# Autodesk Inventor assembly: お盆試作2
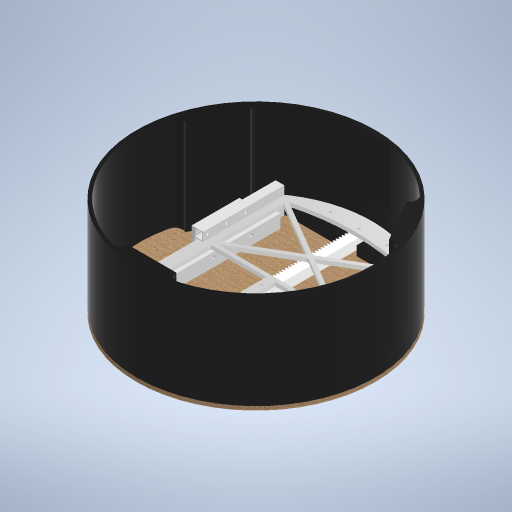
[picture p0: Inventor's stored thumbnail of the model, 512x512]
Saved by Autodesk Inventor 2023 (Build 270158000, 158)
## iProperties
Created: 2022-12-04
Part Number: お盆試作2
Document SubType Name: Assembly
Designer: RiSA
Author: RiSA
## Documents named in this file (9)
- E:\ロボ創\お盆試作2\お盆試作2.iam
- E:\ロボ創\お盆試作2\中間台1.ipt
- E:\ロボ創\お盆試作2\lock1.ipt
- E:\ロボ創\お盆試作2\lock2.ipt
- E:\ロボ創\お盆試作2\allwall.ipt
- E:\ロボ創\お盆試作2\slider.ipt
- E:\ロボ創\お盆試作2\お盆完成予定1.iam
- E:\ロボ創\お盆試作2\stopper.ipt
- E:\ロボ創\お盆試作2\squareEx1.ipt
## Components (11 placed, 8 different names)
1. 中間台1:1 — メイト:1, メイト:2, メイト:3, メイト:4, メイト:5, メイト:6, メイト:7, メイト:8
2. lock1:2 — メイト:1, メイト:2, メイト:3, メイト:9, メイト:10, メイト:11, フラッシュ:1, フラッシュ:2, メイト:19, メイト:20, メイト:21
3. lock2:1 — メイト:4, メイト:5, メイト:6, メイト:12, メイト:13, メイト:14, メイト:16, メイト:17, メイト:18
4. allwall:1 — メイト:7, メイト:8
5. slider:1 — メイト:9, メイト:10, メイト:11
6. slider:2 — メイト:12, メイト:13, メイト:14, メイト:15
7. お盆完成予定1:1 [sub-assembly] — メイト:15, フラッシュ:1, フラッシュ:2
8. stopper:1 — メイト:16, メイト:17, メイト:18, メイト:25, メイト:26
9. stopper:2 — メイト:19, メイト:20, メイト:21, メイト:22, メイト:23, メイト:24
10. squareEx1:1 — メイト:22, メイト:23, メイト:24
11. squareEx1:2 — メイト:25, メイト:26
## Relationships (28: Mate 26, Flush 2)
- メイト:1 [Mate]: 中間台1:1 ↔ lock1:2
- メイト:2 [Mate]: 中間台1:1 ↔ lock1:2
- メイト:3 [Mate]: 中間台1:1 ↔ lock1:2
- メイト:4 [Mate]: 中間台1:1 ↔ lock2:1
- メイト:5 [Mate]: 中間台1:1 ↔ lock2:1
- メイト:6 [Mate]: 中間台1:1 ↔ lock2:1
- メイト:7 [Mate]: 中間台1:1 ↔ allwall:1
- メイト:8 [Mate]: 中間台1:1 ↔ allwall:1
- メイト:9 [Mate]: lock1:2 ↔ slider:1
- メイト:10 [Mate]: lock1:2 ↔ slider:1
- メイト:11 [Mate]: lock1:2 ↔ slider:1
- メイト:12 [Mate]: lock2:1 ↔ slider:2
- メイト:13 [Mate]: lock2:1 ↔ slider:2
- メイト:14 [Mate]: lock2:1 ↔ slider:2
- メイト:15 [Mate]: slider:2 ↔ お盆完成予定1:1
- フラッシュ:1 [Flush]: lock1:2 ↔ お盆完成予定1:1
- フラッシュ:2 [Flush]: lock1:2 ↔ お盆完成予定1:1
- メイト:16 [Mate]: lock2:1 ↔ stopper:1
- メイト:17 [Mate]: lock2:1 ↔ stopper:1
- メイト:18 [Mate]: lock2:1 ↔ stopper:1
- メイト:19 [Mate]: lock1:2 ↔ stopper:2
- メイト:20 [Mate]: lock1:2 ↔ stopper:2
- メイト:21 [Mate]: lock1:2 ↔ stopper:2
- メイト:22 [Mate]: stopper:2 ↔ squareEx1:1
- メイト:23 [Mate]: stopper:2 ↔ squareEx1:1
- メイト:24 [Mate]: stopper:2 ↔ squareEx1:1
- メイト:25 [Mate]: stopper:1 ↔ squareEx1:2
- メイト:26 [Mate]: stopper:1 ↔ squareEx1:2
